# Autodesk Inventor assembly: Montagem Virabrequim
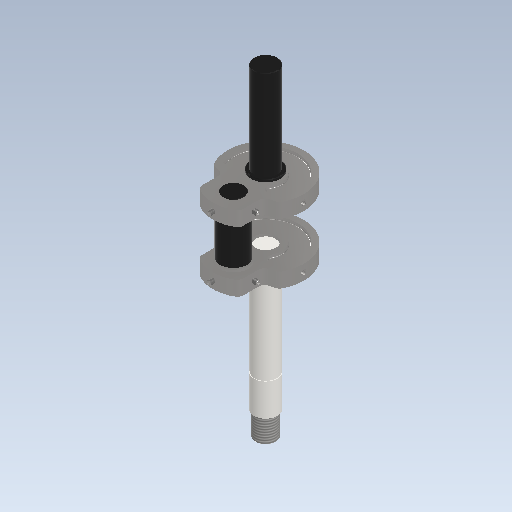
[picture p0: Inventor's stored thumbnail of the model, 512x512]
Saved by Autodesk Inventor 2021 (Build 250183000, 183)
## iProperties
Category: 10
Company: UFABC
Created: 2021-07-26
Document SubType Name: Assembly
Designer: Giovanni
User Status: 1:4
Description: 3
Author: Giovanni Rodrigues Dias
Title: Montagem Virabrequim
Keywords: 4
Revision Number: 01
## Documents named in this file (6)
- C:\Users\irineu\Documents\Inventor\MotorRadial7\Conjunto_Virabrequim.iam
- C:\Users\irineu\Documents\Inventor\MotorRadial7\Contrapeso.ipt
- C:\Users\irineu\Documents\Inventor\MotorRadial7\Eixo Central.ipt
- C:\Users\irineu\Documents\Inventor\MotorRadial7\Eixo Frontal.ipt
- C:\Users\irineu\Documents\Inventor\MotorRadial7\Eixo Traseiro.ipt
- C:\Users\irineu\Documents\Inventor\Content Center Files\R2021\pt-BR\DIN 913\DIN 913 - M8 x 25.ipt
## Components (17 placed, 5 different names)
1. Contrapeso:1 — Alinhado:1, Alinhado:2, Alinhado:3, Inserir:1, Inserir:3, Coincidente:2, Coincidente:4
2. Eixo Central:1 — Inserir:1, Inserir:2, Tangente:1, Tangente:2
3. Contrapeso:2 — Inserir:2, Coincidente:1, Inserir:4, Coincidente:3, Coincidente:5
4. Eixo Frontal:1 — Inserir:3, Alinhado:4, Tangente:3
5. Eixo Traseiro:1 — Inserir:4, Tangente:4
6. DIN 913 M8 x 25:1 — Coincidente:2, Tangente:1
7. DIN 913 M8 x 25:2 — Coincidente:3, Tangente:2
8. DIN 913 M8 x 25:5
9. DIN 913 M8 x 25:6
10. DIN 913 M8 x 25:7
11. DIN 913 M8 x 25:8
12. DIN 913 M8 x 25:3 — Coincidente:4, Tangente:3
13. DIN 913 M8 x 25:4 — Coincidente:5, Tangente:4
14. DIN 913 M8 x 25:9
15. DIN 913 M8 x 25:10
16. DIN 913 M8 x 25:11
17. DIN 913 M8 x 25:12
## Component patterns: (3 elements, first: DIN 913 M8 x 25:1 + DIN 913 M8 x 25:2), (3 elements, first: DIN 913 M8 x 25:3 + DIN 913 M8 x 25:4)
## Relationships (17: Mate 5, Flush 4, Insert 4, Tangent 4)
- Alinhado:1 [Flush]: Contrapeso:1
- Alinhado:2 [Flush]: Contrapeso:1
- Alinhado:3 [Flush]: Contrapeso:1
- Inserir:1: Contrapeso:1 ↔ Eixo Central:1
- Inserir:2: Eixo Central:1 ↔ Contrapeso:2
- Coincidente:1 [Mate]: Contrapeso:2
- Inserir:3: Contrapeso:1 ↔ Eixo Frontal:1
- Alinhado:4 [Flush]: Eixo Frontal:1
- Inserir:4 (-3.3 mm): Contrapeso:2 ↔ Eixo Traseiro:1
- Coincidente:2 [Mate]: Contrapeso:1 ↔ DIN 913 M8 x 25:1
- Coincidente:3 [Mate]: Contrapeso:2 ↔ DIN 913 M8 x 25:2
- Tangente:1: Eixo Central:1 ↔ DIN 913 M8 x 25:1
- Tangente:2: Eixo Central:1 ↔ DIN 913 M8 x 25:2
- Coincidente:4 [Mate]: Contrapeso:1 ↔ DIN 913 M8 x 25:3
- Coincidente:5 [Mate]: Contrapeso:2 ↔ DIN 913 M8 x 25:4
- Tangente:3: Eixo Frontal:1 ↔ DIN 913 M8 x 25:3
- Tangente:4: Eixo Traseiro:1 ↔ DIN 913 M8 x 25:4
